# Autodesk Inventor assembly: Electronica
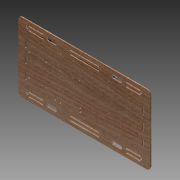
[picture p0: Inventor's stored thumbnail of the model, 180x180]
Saved by Autodesk Inventor 2015 (Build 190159000, 159)
## iProperties
Created: 2015-12-19
Part Number: Electronica
Document SubType Name: Assembly
Designer: david
Author: david
## Documents named in this file (7)
- Z:\gip\Inventor\generatie 7\Frame\Electronica\Electronica.iam
- Z:\gip\Inventor\generatie 7\Frame\Electronica\plaat.ipt
- Z:\gip\Inventor\generatie 7\Frame\Electronica\printplaat\printplaat.iam
- Z:\gip\Inventor\generatie 7\Frame\Electronica\Arduino nano\Assembly.iam
- Z:\gip\Inventor\generatie 7\Frame\Electronica\Baterij\Baterij.ipt.iam
- Z:\gip\Inventor\generatie 7\Frame\Electronica\relais\Relais.iam
- Baterij.ipt
## Components (5 placed, 5 different names)
1. plaat:1 — Mate:2, Flush:1, Flush:2, Mate:7, Mate:8, Mate:9, Angle:1
2. Baterij.ipt:1 [sub-assembly] — Flush:2, Mate:7
3. printplaat:1 [sub-assembly] — Mate:2, Flush:1, Mate:3, Mate:4, Mate:5
4. Assembly:1 [sub-assembly] — Mate:3, Mate:4, Mate:5
5. Relais:1 [sub-assembly] — Mate:8, Mate:9, Angle:1
## Relationships (11: Mate 8, Flush 2, Angle 1)
- Mate:2 (2 mm): plaat:1 ↔ printplaat:1
- Flush:1 (75 mm): plaat:1 ↔ printplaat:1
- Mate:3: printplaat:1 ↔ Assembly:1
- Mate:4: printplaat:1 ↔ Assembly:1
- Mate:5: printplaat:1 ↔ Assembly:1
- [Mate]: plaat:1 ↔ Baterij.ipt:1
- Flush:2 (5 mm): plaat:1 ↔ Baterij.ipt:1
- Mate:7 (-20 mm): plaat:1 ↔ Baterij.ipt:1
- Mate:8: plaat:1 ↔ Relais:1
- Mate:9 (2 mm): plaat:1 ↔ Relais:1
- Angle:1 (0 deg): plaat:1 ↔ Relais:1
